# Autodesk Inventor assembly: halfcut-60t-gear
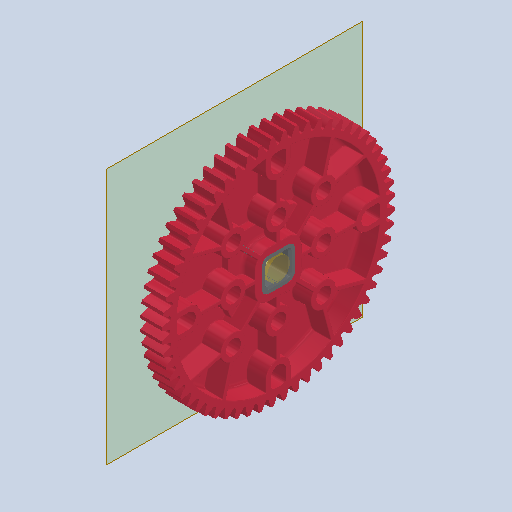
[picture p0: Inventor's stored thumbnail of the model, 512x512]
Saved by Autodesk Inventor 2025.2 (Build 292293000, 293)
## iProperties
Created: 2025-07-20
Part Number: halfcut-60t-gear
Document SubType Name: Assembly
Designer: Exortions
Author: Exortions
## Documents named in this file (3)
- C:\3284b-cad-2025\Library\Custom Parts\halfcut-60t-gear.iam
- C:\3284b-cad-2025\Library\VEX-CAD-Inventor-1.4.2\Motion\Gears\HS Gear\HS 60T Gear, No Insert.iam
- C:\3284b-cad-2025\Library\VEX-CAD-Inventor-1.4.2\Motion\Gears\HS Gear.iam
## Components (1 placed, 1 different names)
1. HS 60T Gear, No Insert:1 [sub-assembly] — Mate:1, Angle:1
## Relationships (2: Mate 1, Angle 1)
- Mate:1: HS 60T Gear, No Insert:1
- Angle:1 (0 deg): HS 60T Gear, No Insert:1
